# Autodesk Inventor assembly: Final_Reduccion
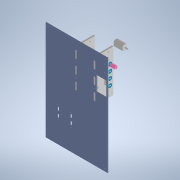
[picture p0: Inventor's stored thumbnail of the model, 180x180]
Saved by Autodesk Inventor 2022 (Build 260153000, 153)
## iProperties
Created: 2022-03-13
Part Number: Final_Reduccion
Document SubType Name: Assembly
Designer: katha
Author: katha
## Documents named in this file (14)
- C:\Users\katha\OneDrive\Escritorio\Mini_Proyecto_Diseno\Diseno_18012\Modelo_MPD\Final_Reduccion.iam
- C:\Users\katha\OneDrive\Escritorio\Mini_Proyecto_Diseno\Diseno_18012\Modelo_MPD\eje1_n.ipt
- C:\Users\katha\OneDrive\Escritorio\Mini_Proyecto_Diseno\Diseno_18012\Modelo_MPD\eje2_n.ipt
- C:\Users\katha\OneDrive\Escritorio\Mini_Proyecto_Diseno\Diseno_18012\Modelo_MPD\eje3_n.ipt
- C:\Users\katha\OneDrive\Escritorio\Mini_Proyecto_Diseno\Diseno_18012\Modelo_MPD\engranaje40.ipt
- C:\Users\katha\OneDrive\Escritorio\Mini_Proyecto_Diseno\Diseno_18012\Modelo_MPD\engranaje10.ipt
- C:\Users\katha\OneDrive\Escritorio\Mini_Proyecto_Diseno\Diseno_18012\Modelo_MPD\hombro_nuevo.ipt
- C:\Users\katha\OneDrive\Escritorio\Mini_Proyecto_Diseno\Diseno_18012\Modelo_MPD\eje4_n.ipt
- C:\Users\katha\OneDrive\Escritorio\Mini_Proyecto_Diseno\Diseno_18012\Modelo_MPD\Base_proyecto.ipt
- C:\Users\katha\OneDrive\Escritorio\Mini_Proyecto_Diseno\Diseno_18012\Modelo_MPD\caja_2_Lateral.ipt
- C:\Users\katha\OneDrive\Escritorio\Mini_Proyecto_Diseno\Diseno_18012\Modelo_MPD\Rodamiento_Ejes.ipt
- C:\Users\katha\OneDrive\Escritorio\Mini_Proyecto_Diseno\Diseno_18012\Modelo_MPD\Acople_Motor_.ipt
- C:\Users\katha\OneDrive\Escritorio\Mini_Proyecto_Diseno\Diseno_18012\Modelo_MPD\sujetador_motor.ipt
- C:\Users\katha\OneDrive\Escritorio\Mini_Proyecto_Diseno\Diseno_18012\Modelo_MPD\motor_12v.ipt
## Components (28 placed, 13 different names)
1. eje1_n:1 — Mate:1, Mate:2, Mate:3, Mate:4, Mate:5, Flush:1, Mate:45, Mate:46, Flush:21
2. eje2_n:1 — Flush:1, Mate:8, Mate:9, Mate:10, Flush:4, Mate:12, Mate:13, Mate:43, Mate:44
3. engranaje40:1 — Mate:4, Mate:5, Mate:6
4. hombro_nuevo:1 — Mate:1, Mate:2, Mate:3, Mate:6
5. hombro_nuevo:2 — Mate:8, Mate:9, Mate:10, Flush:2, Flush:3, Mate:11
6. engranaje10:1 — Flush:2, Flush:3, Mate:11, Mate:14
7. eje3_n:1 — Flush:4, Mate:15, Mate:16, Mate:17, Mate:19, Mate:20, Flush:7, Mate:41, Flush:20, Mate:42
8. engranaje40:2 — Mate:12, Mate:13, Mate:14
9. hombro_nuevo:3 — Mate:15, Mate:16, Mate:17, Mate:21
10. engranaje10:2 — Flush:5, Flush:6, Mate:18, Mate:19, Mate:20, Mate:21
11. engranaje40:3 — Flush:5, Flush:6, Mate:18
12. eje4_n:1 — Mate:22, Mate:23, Mate:24, Flush:7, Mate:25, Mate:26, Mate:39, Flush:19, Mate:40, Mate:47, Mate:48
13. hombro_nuevo:4 — Mate:22, Mate:23, Mate:24, Mate:27
14. engranaje10:3 — Mate:25, Mate:26, Mate:27
15. Base_proyecto:1 — Mate:28, Mate:29, Flush:8, Mate:30, Flush:22
16. caja_2_Lateral:1 — Mate:28, Mate:29, Flush:8, Flush:9, Flush:10, Mate:31, Mate:32, Mate:33, Mate:34, Flush:15, Flush:16, Flush:17, Flush:18
17. caja_2_Lateral:2 — Flush:9, Flush:10, Mate:30, Mate:35, Mate:36, Mate:37, Mate:38, Flush:11, Flush:12, Flush:13, Flush:14
18. Rodamiento_Ejes:1 — Mate:31, Flush:15, Flush:19, Mate:40
19. Rodamiento_Ejes:2 — Mate:32, Flush:16, Mate:41, Flush:20, Mate:42
20. Rodamiento_Ejes:3 — Mate:33, Flush:17, Mate:43, Mate:44
21. Rodamiento_Ejes:4 — Mate:34, Flush:18, Mate:45, Mate:46
22. Rodamiento_Ejes:5 — Mate:38, Flush:11, Flush:21
23. Rodamiento_Ejes:6 — Mate:37, Flush:12
24. Rodamiento_Ejes:7 — Mate:36, Flush:13
25. Rodamiento_Ejes:8 — Mate:35, Flush:14, Mate:39
26. Acople_Motor_:1 — Mate:47, Mate:48
27. sujetador_motor:1 — Flush:22
28. motor_12v:1 — Flush:23
## Relationships (70: Mate 47, Flush 23)
- Mate:1 (0.45 mm): eje1_n:1 ↔ hombro_nuevo:1
- Mate:2 (0.45 mm): eje1_n:1 ↔ hombro_nuevo:1
- Mate:3: eje1_n:1 ↔ hombro_nuevo:1
- Mate:4 (0.45 mm): eje1_n:1 ↔ engranaje40:1
- Mate:5 (0.45 mm): eje1_n:1 ↔ engranaje40:1
- Mate:6: engranaje40:1 ↔ hombro_nuevo:1
- Flush:1: eje1_n:1 ↔ eje2_n:1
- Mate:8 (0.45 mm): eje2_n:1 ↔ hombro_nuevo:2
- Mate:9 (0.45 mm): eje2_n:1 ↔ hombro_nuevo:2
- Mate:10: eje2_n:1 ↔ hombro_nuevo:2
- Flush:2: hombro_nuevo:2 ↔ engranaje10:1
- Flush:3: hombro_nuevo:2 ↔ engranaje10:1
- Mate:11: hombro_nuevo:2 ↔ engranaje10:1
- Flush:4: eje2_n:1 ↔ eje3_n:1
- Mate:12 (0.45 mm): eje2_n:1 ↔ engranaje40:2
- Mate:13 (0.45 mm): eje2_n:1 ↔ engranaje40:2
- Mate:14: engranaje10:1 ↔ engranaje40:2
- Mate:15 (0.45 mm): eje3_n:1 ↔ hombro_nuevo:3
- Mate:16 (0.45 mm): eje3_n:1 ↔ hombro_nuevo:3
- Mate:17: eje3_n:1 ↔ hombro_nuevo:3
- Flush:5: engranaje10:2 ↔ engranaje40:3
- Flush:6: engranaje10:2 ↔ engranaje40:3
- Mate:18: engranaje10:2 ↔ engranaje40:3
- Mate:19 (0.45 mm): eje3_n:1 ↔ engranaje10:2
- Mate:20 (0.45 mm): eje3_n:1 ↔ engranaje10:2
- Mate:21: hombro_nuevo:3 ↔ engranaje10:2
- Mate:22 (0.45 mm): eje4_n:1 ↔ hombro_nuevo:4
- Mate:23 (0.45 mm): eje4_n:1 ↔ hombro_nuevo:4
- Mate:24: eje4_n:1 ↔ hombro_nuevo:4
- Flush:7: eje3_n:1 ↔ eje4_n:1
- Mate:25 (0.45 mm): eje4_n:1 ↔ engranaje10:3
- Mate:26 (0.45 mm): eje4_n:1 ↔ engranaje10:3
- Mate:27: hombro_nuevo:4 ↔ engranaje10:3
- Mate:28: Base_proyecto:1 ↔ caja_2_Lateral:1
- Mate:29: Base_proyecto:1 ↔ caja_2_Lateral:1
- Flush:8: Base_proyecto:1 ↔ caja_2_Lateral:1
- Flush:9: caja_2_Lateral:1 ↔ caja_2_Lateral:2
- Flush:10: caja_2_Lateral:1 ↔ caja_2_Lateral:2
- Mate:30: Base_proyecto:1 ↔ caja_2_Lateral:2
- Mate:31: caja_2_Lateral:1 ↔ Rodamiento_Ejes:1
- Mate:32: caja_2_Lateral:1 ↔ Rodamiento_Ejes:2
- Mate:33: caja_2_Lateral:1 ↔ Rodamiento_Ejes:3
- Mate:34: caja_2_Lateral:1 ↔ Rodamiento_Ejes:4
- Mate:35: caja_2_Lateral:2 ↔ Rodamiento_Ejes:8
- Mate:36: caja_2_Lateral:2 ↔ Rodamiento_Ejes:7
- Mate:37: caja_2_Lateral:2 ↔ Rodamiento_Ejes:6
- Mate:38: caja_2_Lateral:2 ↔ Rodamiento_Ejes:5
- Flush:11 (0.1 mm): caja_2_Lateral:2 ↔ Rodamiento_Ejes:5
- Flush:12 (0.1 mm): caja_2_Lateral:2 ↔ Rodamiento_Ejes:6
- Flush:13 (-0.1 mm): caja_2_Lateral:2 ↔ Rodamiento_Ejes:7
- Flush:14 (-0.1 mm): caja_2_Lateral:2 ↔ Rodamiento_Ejes:8
- Flush:15 (0.1 mm): caja_2_Lateral:1 ↔ Rodamiento_Ejes:1
- Flush:16 (0.1 mm): caja_2_Lateral:1 ↔ Rodamiento_Ejes:2
- Flush:17 (0.1 mm): caja_2_Lateral:1 ↔ Rodamiento_Ejes:3
- Flush:18 (0.1 mm): caja_2_Lateral:1 ↔ Rodamiento_Ejes:4
- Mate:39 (0.45 mm): eje4_n:1 ↔ Rodamiento_Ejes:8
- Flush:19: eje4_n:1 ↔ Rodamiento_Ejes:1
- Mate:40 (0.45 mm): eje4_n:1 ↔ Rodamiento_Ejes:1
- Mate:41 (0.45 mm): eje3_n:1 ↔ Rodamiento_Ejes:2
- Flush:20: eje3_n:1 ↔ Rodamiento_Ejes:2
- Mate:42 (0.45 mm): eje3_n:1 ↔ Rodamiento_Ejes:2
- Mate:43 (0.45 mm): eje2_n:1 ↔ Rodamiento_Ejes:3
- Mate:44 (0.45 mm): eje2_n:1 ↔ Rodamiento_Ejes:3
- Mate:45 (0.45 mm): eje1_n:1 ↔ Rodamiento_Ejes:4
- Mate:46 (0.45 mm): eje1_n:1 ↔ Rodamiento_Ejes:4
- Flush:21: eje1_n:1 ↔ Rodamiento_Ejes:5
- Mate:47: eje4_n:1 ↔ Acople_Motor_:1
- Mate:48 (0.4 mm): eje4_n:1 ↔ Acople_Motor_:1
- Flush:22: Base_proyecto:1 ↔ sujetador_motor:1
- Flush:23: motor_12v:1
